# Autodesk Inventor assembly: s-assy-gripper_tentioner
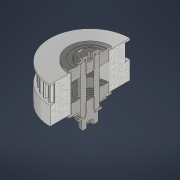
[picture p0: Inventor's stored thumbnail of the model, 180x180]
Saved by Autodesk Inventor 2022 (Build 260153000, 153)
## iProperties
Created: 2021-08-06
Part Number: s-assy-gripper_tentioner
Document SubType Name: Assembly
Designer: yuta0
Mass: 598.977 g
Surface Area: 2161.2 cm^2
Volume: 259.929 cm^3
Density: 2.30439 g/cm^3
Author: yuta0
## Documents named in this file (8)
- C:\Users\yuta0\Documents\GitHub\catchrobo_hardware\assy-robot\s-assy-gripper_tentioner.iam
- C:\Users\yuta0\Documents\GitHub\catchrobo_hardware\assy-robot\base36.ipt
- C:\Users\yuta0\Documents\GitHub\catchrobo_hardware\assy-robot\FL688ZZ.ipt
- C:\Users\yuta0\Documents\GitHub\catchrobo_hardware\assy-robot\CB4-6.ipt
- C:\Users\yuta0\Documents\GitHub\catchrobo_hardware\assy-robot\CC-0814-05.ipt
- C:\Users\yuta0\Documents\GitHub\catchrobo_hardware\assy-robot\WSJ-STN-M4.ipt
- C:\Users\yuta0\Documents\GitHub\catchrobo_hardware\assy-robot\CBSTSR4-6.ipt
- C:\Users\yuta0\Documents\GitHub\catchrobo_hardware\assy-robot\SFHRW8-20-M4-N4_s.ipt
## Components (9 placed, 7 different names)
1. CC-0814-05:1 — メイト:38, メイト:39, メイト:125
2. FL688ZZ:2 — メイト:29, メイト:30, メイト:39, メイト:132
3. WSJ-STN-M4:2 — メイト:87, メイト:125, メイト:127, メイト:128
4. CB4-6:8 — メイト:87, メイト:128
5. CBSTSR4-6:3 — メイト:124, メイト:129, メイト:130
6. WSJ-STN-M4:1 — メイト:124, メイト:130, メイト:131, メイト:133
7. FL688ZZ:1 — メイト:26, メイト:38, メイト:129, メイト:131, メイト:134
8. base36:1 — メイト:26, メイト:29, メイト:30, メイト:127, メイト:134
9. SFHRW8-20-M4-N4_s:1 — メイト:132, メイト:133
## Relationships (16: Mate 16)
- メイト:26 [Mate]: FL688ZZ:1 ↔ base36:1
- メイト:29 [Mate]: FL688ZZ:2 ↔ base36:1
- メイト:30 [Mate]: FL688ZZ:2 ↔ base36:1
- メイト:38 [Mate]: CC-0814-05:1 ↔ FL688ZZ:1
- メイト:39 [Mate]: CC-0814-05:1 ↔ FL688ZZ:2
- メイト:87 [Mate]: WSJ-STN-M4:2 ↔ CB4-6:8
- メイト:124 [Mate]: CBSTSR4-6:3 ↔ WSJ-STN-M4:1
- メイト:125 [Mate] (2 mm): CC-0814-05:1 ↔ WSJ-STN-M4:2
- メイト:127 [Mate]: WSJ-STN-M4:2 ↔ base36:1
- メイト:128 [Mate]: WSJ-STN-M4:2 ↔ CB4-6:8
- メイト:129 [Mate]: CBSTSR4-6:3 ↔ FL688ZZ:1
- メイト:130 [Mate]: CBSTSR4-6:3 ↔ WSJ-STN-M4:1
- メイト:131 [Mate]: WSJ-STN-M4:1 ↔ FL688ZZ:1
- メイト:132 [Mate]: FL688ZZ:2 ↔ SFHRW8-20-M4-N4_s:1
- メイト:133 [Mate]: WSJ-STN-M4:1 ↔ SFHRW8-20-M4-N4_s:1
- メイト:134 [Mate]: FL688ZZ:1 ↔ base36:1
